# Autodesk Inventor assembly: ShoulderLeft
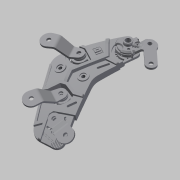
[picture p0: Inventor's stored thumbnail of the model, 180x180]
Saved by Autodesk Inventor 2015 SP1 (Build 190203100, 203)
## iProperties
Created: 2016-10-02
Part Number: ShoulderLeft
Document SubType Name: Assembly
Designer: Val
Author: Val
## Documents named in this file (7)
- C:\Users\Val\Desktop\ExoGit\elysium-max-exoskeleton\src\Assemblies\ShoulderRight.iam
- C:\Users\Val\Desktop\ExoGit\elysium-max-exoskeleton\src\ShoulderCogLarge.ipt
- C:\Users\Val\Desktop\ExoGit\elysium-max-exoskeleton\src\ShoulderCogSmall.ipt
- C:\Users\Val\Desktop\ExoGit\elysium-max-exoskeleton\src\BackConnector.ipt
- C:\Users\Val\Desktop\ExoGit\elysium-max-exoskeleton\src\BackSideConnector.ipt
- C:\Users\Val\Desktop\ExoGit\elysium-max-exoskeleton\src\Assemblies\ShoulderConnector.iam
- C:\Users\Val\Desktop\ExoGit\elysium-max-exoskeleton\src\ShoulderRight.ipt
## Components (10 placed, 6 different names)
1. ShoulderCogLarge:1 — Mate:19, Mate:20, Mate:22
2. ShoulderCogSmall:1 — Mate:14, Mate:29, Mate:30, Mate:31
3. ShoulderCogSmall:2 — Mate:16, Mate:26, Mate:27
4. ShoulderCogSmall:3 — Mate:18, Mate:23, Mate:24
5. BackConnector:1 — Mate:14, Mate:31, Mate:32
6. BackSideConnector:1 — Mate:11, Mate:12
7. BackConnector:2 — Mate:16, Mate:28
8. BackConnector:3 — Mate:18, Mate:25
9. ShoulderConnectorSplit:1 [sub-assembly] — Mate:11, Mate:12, Mate:21, Mate:22
10. ShoulderRight:1 — Mate:19, Mate:20, Mate:21, Mate:23, Mate:24, Mate:25, Mate:26, Mate:27, Mate:28, Mate:29, Mate:30, Mate:32
## Relationships (19: Mate 19)
- Mate:11: BackSideConnector:1 ↔ ShoulderConnectorSplit:1
- Mate:12: BackSideConnector:1 ↔ ShoulderConnectorSplit:1
- Mate:14: ShoulderCogSmall:1 ↔ BackConnector:1
- Mate:16: ShoulderCogSmall:2 ↔ BackConnector:2
- Mate:18: ShoulderCogSmall:3 ↔ BackConnector:3
- Mate:19: ShoulderCogLarge:1 ↔ ShoulderRight:1
- Mate:20: ShoulderCogLarge:1 ↔ ShoulderRight:1
- Mate:21: ShoulderConnectorSplit:1 ↔ ShoulderRight:1
- Mate:22: ShoulderCogLarge:1 ↔ ShoulderConnectorSplit:1
- Mate:23: ShoulderCogSmall:3 ↔ ShoulderRight:1
- Mate:24: ShoulderCogSmall:3 ↔ ShoulderRight:1
- Mate:25: BackConnector:3 ↔ ShoulderRight:1
- Mate:26: ShoulderCogSmall:2 ↔ ShoulderRight:1
- Mate:27: ShoulderCogSmall:2 ↔ ShoulderRight:1
- Mate:28: BackConnector:2 ↔ ShoulderRight:1
- Mate:29: ShoulderCogSmall:1 ↔ ShoulderRight:1
- Mate:30: ShoulderCogSmall:1 ↔ ShoulderRight:1
- Mate:31: ShoulderCogSmall:1 ↔ BackConnector:1
- Mate:32: BackConnector:1 ↔ ShoulderRight:1
